# Autodesk Inventor assembly: MotorMount_Mount
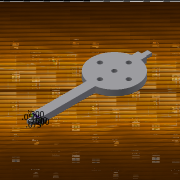
[picture p0: Inventor's stored thumbnail of the model, 180x180]
Saved by Autodesk Inventor 2017 (Build 210142000, 142)
## iProperties
Created: 2017-01-13
Part Number: MotorMount_Mount
Document SubType Name: Assembly
Designer: David Kopala
Author: David Kopala
## Documents named in this file (3)
- Z:\Documents\Drone\Drone\3D Models\Project\Chasis_03\PrinterVersions\ReadyFiles\MotorMount_Mount.iam
- Z:\Documents\Drone\Drone\3D Models\Project\Chasis_03\MotorMount_Part.ipt
- Z:\Documents\Drone\Drone\3D Models\Project\Chasis_03\PrinterVersions\MotorMount_Insert\Part1.ipt
## Components (3 placed, 2 different names)
1. MotorMount_Part:1 — Flush:1, Mate:1, Flush:2, Flush:3, Mate:2, Flush:4, Flush:5
2. Part1:1 — Flush:1, Mate:1, Flush:2, Flush:3
3. Part1:2 — Mate:2, Flush:4, Flush:5
## Relationships (7: Flush 5, Mate 2)
- Flush:1: MotorMount_Part:1 ↔ Part1:1
- Mate:1: MotorMount_Part:1 ↔ Part1:1
- Flush:2 (1.27 mm): MotorMount_Part:1 ↔ Part1:1
- Flush:3 (1.905 mm): MotorMount_Part:1 ↔ Part1:1
- Mate:2: MotorMount_Part:1 ↔ Part1:2
- Flush:4 (1.27 mm): MotorMount_Part:1 ↔ Part1:2
- Flush:5 (1.905 mm): MotorMount_Part:1 ↔ Part1:2
